# Autodesk Inventor assembly: MicroSD Card in Reader
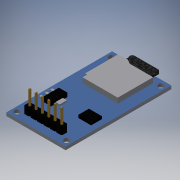
[picture p0: Inventor's stored thumbnail of the model, 180x180]
Saved by Autodesk Inventor 2016 (Build 200138000, 138)
## iProperties
Created: 2015-11-27
Part Number: MicroSD Card in Reader
Document SubType Name: Assembly
Designer: Spooner
Author: Spooner
## Documents named in this file (4)
- C:\Users\Spooner\Documents\GY81 Logger\3D Models\MicroSD Card in Reader.iam
- C:\Users\Spooner\Documents\GY81 Logger\3D Models\MicroSD Card Reader.ipt
- C:\Users\Spooner\Documents\GY81 Logger\3D Models\MicroSD Card.ipt
- C:\Users\Spooner\Documents\GY81 Logger\3D Models\6 Short Male Headers.ipt
## Components (3 placed, 3 different names)
1. MicroSD Card Reader:1 — Mate:1, Mate:2, Flush:1, Mate:3, Mate:4, Mate:5
2. MicroSD Card:1 — Mate:1, Mate:2, Flush:1
3. 6 Short Male Headers:1 — Mate:3, Mate:4, Mate:5
## Relationships (6: Mate 5, Flush 1)
- Mate:1: MicroSD Card Reader:1 ↔ MicroSD Card:1
- Mate:2: MicroSD Card Reader:1 ↔ MicroSD Card:1
- Flush:1 (-2.6797 mm): MicroSD Card Reader:1 ↔ MicroSD Card:1
- Mate:3: MicroSD Card Reader:1 ↔ 6 Short Male Headers:1
- Mate:4: MicroSD Card Reader:1 ↔ 6 Short Male Headers:1
- Mate:5: MicroSD Card Reader:1 ↔ 6 Short Male Headers:1
